# Autodesk Inventor assembly: Asem
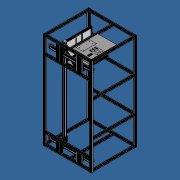
[picture p0: Inventor's stored thumbnail of the model, 180x180]
Saved by Autodesk Inventor 2020 (Build 240168000, 168)
## iProperties
Created: 2021-02-24
Part Number: Asem
Document SubType Name: Assembly
Designer: magnarecta
Author: magnarecta
## Documents named in this file (12)
- D:\Document\Github\Eto_Project\Hardware\Asem\Asem.iam
- D:\Document\Github\Eto_Project\Hardware\Parts\MISUMI\HFS6-3030-1500_Autodesk_Inventor_2020_20210225\HFS6-3030-1500.ipt
- D:\Document\Github\Eto_Project\Hardware\Parts\MISUMI\HFS6-3030-690_Autodesk_Inventor_2020_20210225\HFS6-3030-690.ipt
- D:\Document\Github\Eto_Project\Hardware\Asem\CCM_Unit.iam
- D:\Document\Github\Eto_Project\Hardware\Parts\MISUMI\HFS6-3030-223_Autodesk_Inventor_2020_20210225\HFS6-3030-223.ipt
- D:\Document\Github\Eto_Project\Hardware\Parts\MISUMI\HFS6-3030-140_Autodesk_Inventor_2020_20210225\HFS6-3030-140.ipt
- D:\Document\Github\Eto_Project\Hardware\Asem\Display_Unit.iam
- D:\Document\Github\Eto_Project\Hardware\Parts\MISUMI\HFS6-3030-650_Autodesk_Inventor_2020_20210518\HFS6-3030-650.ipt
- D:\Document\Github\Eto_Project\Hardware\Parts\Meviy\Controller_Panel.ipt
- D:\Document\Github\Eto_Project\Hardware\Parts\Grabcad\ac-power-switch-assembly-1.snapshot.2\AC Power Switch Assy.iam
- D:\Document\Github\Eto_Project\Hardware\Parts\Grabcad\mean-well-lrs-350-24-1.snapshot.3\meanwell_lrs-350-24_UPDATED.ipt
- D:\Document\Github\Eto_Project\Hardware\Parts\Grabcad\nema-23-stepper-motors-driver-1.snapshot.7\DM542T Digital Stepper Drive.ipt
## Components (36 placed, 11 different names)
1. HFS6-3030-1500:1 — フラッシュ:1, フラッシュ:2, フラッシュ:5, メイト:1, フラッシュ:6, フラッシュ:7, フラッシュ:9, フラッシュ:10, フラッシュ:25, メイト:20
2. HFS6-3030-1500:2 — フラッシュ:2, フラッシュ:5, メイト:1, フラッシュ:8, メイト:3, メイト:4, フラッシュ:11, フラッシュ:12, メイト:12, メイト:13, フラッシュ:26, メイト:28, メイト:29, フラッシュ:52, フラッシュ:53
3. HFS6-3030-1500:3 — フラッシュ:3, フラッシュ:4, フラッシュ:8, メイト:5, フラッシュ:13, フラッシュ:14, メイト:6, フラッシュ:15, フラッシュ:16, メイト:32, メイト:33, フラッシュ:57, フラッシュ:59
4. HFS6-3030-1500:4 — フラッシュ:1, フラッシュ:3, フラッシュ:4, フラッシュ:6, フラッシュ:7, メイト:27
5. HFS6-3030-690:1 — メイト:3, フラッシュ:9, フラッシュ:10, メイト:15, メイト:18, フラッシュ:33, メイト:19, メイト:30, フラッシュ:61, メイト:36
6. HFS6-3030-690:2 — メイト:4, フラッシュ:11, フラッシュ:12, メイト:11, 角度:1, メイト:14, フラッシュ:28, メイト:31, フラッシュ:55
7. HFS6-3030-690:3 — メイト:5, フラッシュ:13, フラッシュ:14
8. HFS6-3030-690:4 — メイト:6, フラッシュ:15, フラッシュ:16, フラッシュ:54
9. HFS6-3030-650:1 — メイト:34
10. HFS6-3030-650:2
11. HFS6-3030-650:3 — メイト:27
12. HFS6-3030-650:4
13. CCM_Unit:1 [sub-assembly] — メイト:11, 角度:1, フラッシュ:27, フラッシュ:34, フラッシュ:36
14. HFS6-3030-690:5 — メイト:12, フラッシュ:25, メイト:14, フラッシュ:43, メイト:21
15. HFS6-3030-690:6 — メイト:13, フラッシュ:26, メイト:15, フラッシュ:35
16. HFS6-3030-223:1 — フラッシュ:31, フラッシュ:32, メイト:17, メイト:18, フラッシュ:47
17. HFS6-3030-223:2 — フラッシュ:31, フラッシュ:32, メイト:17, フラッシュ:33, フラッシュ:34, メイト:20, フラッシュ:44
18. HFS6-3030-223:3 — フラッシュ:29, フラッシュ:30, メイト:16, フラッシュ:46
19. HFS6-3030-223:4 — フラッシュ:29, フラッシュ:30, メイト:16, メイト:19, フラッシュ:35, フラッシュ:36, フラッシュ:45
20. HFS6-3030-140:1 — フラッシュ:37, フラッシュ:42, メイト:21, フラッシュ:44
21. HFS6-3030-140:2 — フラッシュ:37, フラッシュ:38, フラッシュ:41, フラッシュ:42, フラッシュ:43, フラッシュ:46
22. HFS6-3030-140:3 — フラッシュ:38, フラッシュ:39, フラッシュ:40, フラッシュ:41, フラッシュ:47
23. HFS6-3030-140:4 — フラッシュ:39, フラッシュ:40, フラッシュ:45
24. Display_Unit:1 [sub-assembly]
25. HFS6-3030-650:5 — メイト:28, フラッシュ:53, フラッシュ:58
26. HFS6-3030-650:6 — メイト:29, フラッシュ:52, フラッシュ:60
27. HFS6-3030-650:7 — メイト:30, フラッシュ:54, フラッシュ:56, メイト:35
28. HFS6-3030-650:8 — メイト:31, フラッシュ:55, フラッシュ:56
29. HFS6-3030-690:7 — メイト:32, フラッシュ:59, フラッシュ:60
30. HFS6-3030-690:8 — メイト:33, フラッシュ:57, フラッシュ:58
31. Controller_Panel:1 — メイト:34, フラッシュ:61, メイト:35, メイト:36, 挿入:1, 挿入:2, 挿入:3, 挿入:4, メイト:37, 挿入:5, 角度:2
32. AC Power Switch Assy:1 [sub-assembly] — 挿入:3, 挿入:4
33. meanwell_lrs-350-24_UPDATED:1 — 挿入:1, 挿入:2
34. DM542T Digital Stepper Drive:1 — メイト:37, 挿入:5
35. DM542T Digital Stepper Drive:2
36. DM542T Digital Stepper Drive:3 — 角度:2
## Component patterns: (3 elements, first: DM542T Digital Stepper Drive:1)
## Relationships (95: Flush 57, Mate 31, Insert 5, Angle 2)
- フラッシュ:1 [Flush]: HFS6-3030-1500:1 ↔ HFS6-3030-1500:4
- フラッシュ:2 [Flush]: HFS6-3030-1500:1 ↔ HFS6-3030-1500:2
- フラッシュ:3 [Flush]: HFS6-3030-1500:3 ↔ HFS6-3030-1500:4
- フラッシュ:4 [Flush]: HFS6-3030-1500:3 ↔ HFS6-3030-1500:4
- フラッシュ:5 [Flush]: HFS6-3030-1500:1 ↔ HFS6-3030-1500:2
- メイト:1 [Mate] (-750 mm): HFS6-3030-1500:1 ↔ HFS6-3030-1500:2
- フラッシュ:6 [Flush]: HFS6-3030-1500:1 ↔ HFS6-3030-1500:4
- フラッシュ:7 [Flush]: HFS6-3030-1500:1 ↔ HFS6-3030-1500:4
- フラッシュ:8 [Flush]: HFS6-3030-1500:2 ↔ HFS6-3030-1500:3
- メイト:3 [Mate]: HFS6-3030-1500:2 ↔ HFS6-3030-690:1
- フラッシュ:9 [Flush]: HFS6-3030-1500:1 ↔ HFS6-3030-690:1
- フラッシュ:10 [Flush]: HFS6-3030-1500:1 ↔ HFS6-3030-690:1
- メイト:4 [Mate]: HFS6-3030-1500:2 ↔ HFS6-3030-690:2
- フラッシュ:11 [Flush]: HFS6-3030-1500:2 ↔ HFS6-3030-690:2
- フラッシュ:12 [Flush]: HFS6-3030-1500:2 ↔ HFS6-3030-690:2
- メイト:5 [Mate]: HFS6-3030-1500:3 ↔ HFS6-3030-690:3
- フラッシュ:13 [Flush]: HFS6-3030-1500:3 ↔ HFS6-3030-690:3
- フラッシュ:14 [Flush]: HFS6-3030-1500:3 ↔ HFS6-3030-690:3
- メイト:6 [Mate]: HFS6-3030-1500:3 ↔ HFS6-3030-690:4
- フラッシュ:15 [Flush]: HFS6-3030-1500:3 ↔ HFS6-3030-690:4
- フラッシュ:16 [Flush]: HFS6-3030-1500:3 ↔ HFS6-3030-690:4
- [Mate]: HFS6-3030-690:1 ↔ HFS6-3030-650:1
- [Flush]: HFS6-3030-690:1 ↔ HFS6-3030-650:1
- [Mate]: HFS6-3030-690:1 ↔ HFS6-3030-650:2
- [Flush]: HFS6-3030-1500:1 ↔ HFS6-3030-650:2
- [Flush]: HFS6-3030-690:1 ↔ HFS6-3030-650:2
- [Flush]: HFS6-3030-1500:2 ↔ HFS6-3030-650:1
- [Mate]: HFS6-3030-690:2 ↔ HFS6-3030-650:3
- [Flush]: HFS6-3030-1500:1 ↔ HFS6-3030-650:3
- [Flush]: HFS6-3030-690:2 ↔ HFS6-3030-650:3
- [Mate]: HFS6-3030-1500:2 ↔ HFS6-3030-650:4
- [Flush]: HFS6-3030-690:2 ↔ HFS6-3030-650:4
- [Flush]: HFS6-3030-1500:2 ↔ HFS6-3030-650:4
- メイト:11 [Mate] (2 mm): HFS6-3030-690:2 ↔ CCM_Unit:1
- 角度:1 [Angle] (0 deg): HFS6-3030-690:2 ↔ CCM_Unit:1
- メイト:12 [Mate]: HFS6-3030-1500:2 ↔ HFS6-3030-690:5
- フラッシュ:25 [Flush]: HFS6-3030-1500:1 ↔ HFS6-3030-690:5
- メイト:13 [Mate]: HFS6-3030-1500:2 ↔ HFS6-3030-690:6
- フラッシュ:26 [Flush]: HFS6-3030-1500:2 ↔ HFS6-3030-690:6
- メイト:14 [Mate] (-200 mm): HFS6-3030-690:2 ↔ HFS6-3030-690:5
- メイト:15 [Mate] (-283 mm): HFS6-3030-690:1 ↔ HFS6-3030-690:6
- フラッシュ:27 [Flush] (-10 mm): CCM_Unit:1
- フラッシュ:28 [Flush] (70 mm): HFS6-3030-690:2
- フラッシュ:29 [Flush]: HFS6-3030-223:3 ↔ HFS6-3030-223:4
- フラッシュ:30 [Flush]: HFS6-3030-223:3 ↔ HFS6-3030-223:4
- メイト:16 [Mate] (20 mm): HFS6-3030-223:3 ↔ HFS6-3030-223:4
- フラッシュ:31 [Flush]: HFS6-3030-223:1 ↔ HFS6-3030-223:2
- フラッシュ:32 [Flush]: HFS6-3030-223:1 ↔ HFS6-3030-223:2
- メイト:17 [Mate] (20 mm): HFS6-3030-223:1 ↔ HFS6-3030-223:2
- メイト:18 [Mate]: HFS6-3030-690:1 ↔ HFS6-3030-223:1
- フラッシュ:33 [Flush]: HFS6-3030-690:1 ↔ HFS6-3030-223:2
- フラッシュ:34 [Flush] (-7.5 mm): CCM_Unit:1 ↔ HFS6-3030-223:2
- メイト:19 [Mate]: HFS6-3030-690:1 ↔ HFS6-3030-223:4
- フラッシュ:35 [Flush]: HFS6-3030-690:6 ↔ HFS6-3030-223:4
- フラッシュ:36 [Flush]: CCM_Unit:1 ↔ HFS6-3030-223:4
- メイト:20 [Mate] (170 mm): HFS6-3030-1500:1 ↔ HFS6-3030-223:2
- フラッシュ:37 [Flush]: HFS6-3030-140:1 ↔ HFS6-3030-140:2
- フラッシュ:38 [Flush]: HFS6-3030-140:2 ↔ HFS6-3030-140:3
- フラッシュ:39 [Flush]: HFS6-3030-140:3 ↔ HFS6-3030-140:4
- フラッシュ:40 [Flush]: HFS6-3030-140:3 ↔ HFS6-3030-140:4
- フラッシュ:41 [Flush]: HFS6-3030-140:2 ↔ HFS6-3030-140:3
- フラッシュ:42 [Flush]: HFS6-3030-140:1 ↔ HFS6-3030-140:2
- フラッシュ:43 [Flush]: HFS6-3030-690:5 ↔ HFS6-3030-140:2
- メイト:21 [Mate]: HFS6-3030-690:5 ↔ HFS6-3030-140:1
- フラッシュ:44 [Flush]: HFS6-3030-223:2 ↔ HFS6-3030-140:1
- フラッシュ:45 [Flush]: HFS6-3030-223:4 ↔ HFS6-3030-140:4
- フラッシュ:46 [Flush]: HFS6-3030-223:3 ↔ HFS6-3030-140:2
- フラッシュ:47 [Flush]: HFS6-3030-223:1 ↔ HFS6-3030-140:3
- メイト:27 [Mate]: HFS6-3030-1500:4 ↔ HFS6-3030-650:3
- メイト:28 [Mate]: HFS6-3030-1500:2 ↔ HFS6-3030-650:5
- メイト:29 [Mate]: HFS6-3030-1500:2 ↔ HFS6-3030-650:6
- フラッシュ:52 [Flush]: HFS6-3030-1500:2 ↔ HFS6-3030-650:6
- フラッシュ:53 [Flush]: HFS6-3030-1500:2 ↔ HFS6-3030-650:5
- メイト:30 [Mate]: HFS6-3030-690:1 ↔ HFS6-3030-650:7
- フラッシュ:54 [Flush]: HFS6-3030-690:4 ↔ HFS6-3030-650:7
- メイト:31 [Mate]: HFS6-3030-690:2 ↔ HFS6-3030-650:8
- フラッシュ:55 [Flush]: HFS6-3030-690:2 ↔ HFS6-3030-650:8
- フラッシュ:56 [Flush]: HFS6-3030-650:7 ↔ HFS6-3030-650:8
- メイト:32 [Mate]: HFS6-3030-1500:3 ↔ HFS6-3030-690:7
- メイト:33 [Mate]: HFS6-3030-1500:3 ↔ HFS6-3030-690:8
- フラッシュ:57 [Flush]: HFS6-3030-1500:3 ↔ HFS6-3030-690:8
- フラッシュ:58 [Flush]: HFS6-3030-650:5 ↔ HFS6-3030-690:8
- フラッシュ:59 [Flush]: HFS6-3030-1500:3 ↔ HFS6-3030-690:7
- フラッシュ:60 [Flush]: HFS6-3030-650:6 ↔ HFS6-3030-690:7
- メイト:34 [Mate]: HFS6-3030-650:1 ↔ Controller_Panel:1
- フラッシュ:61 [Flush]: HFS6-3030-690:1 ↔ Controller_Panel:1
- メイト:35 [Mate]: HFS6-3030-650:7 ↔ Controller_Panel:1
- メイト:36 [Mate]: HFS6-3030-690:1 ↔ Controller_Panel:1
- 挿入:1 [Insert]: Controller_Panel:1 ↔ meanwell_lrs-350-24_UPDATED:1
- 挿入:2 [Insert]: Controller_Panel:1 ↔ meanwell_lrs-350-24_UPDATED:1
- 挿入:3 [Insert]: Controller_Panel:1 ↔ AC Power Switch Assy:1
- 挿入:4 [Insert]: Controller_Panel:1 ↔ AC Power Switch Assy:1
- メイト:37 [Mate]: Controller_Panel:1 ↔ DM542T Digital Stepper Drive:1
- 挿入:5 [Insert]: Controller_Panel:1 ↔ DM542T Digital Stepper Drive:1
- 角度:2 [Angle] (0 deg): Controller_Panel:1 ↔ DM542T Digital Stepper Drive:3
